# Autodesk Inventor assembly: Mount Setup
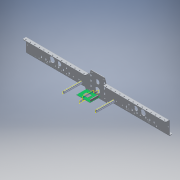
[picture p0: Inventor's stored thumbnail of the model, 180x180]
Saved by Autodesk Inventor 2017 (Build 210142000, 142)
## iProperties
Created: 2017-02-12
Part Number: Mount Setup
Document SubType Name: Assembly
Designer: Roksbot
Author: Roksbot
## Documents named in this file (4)
- C:\Users\Roksbot\Documents\Inventor\FRC ADIS16448\Mount Setup.iam
- C:\Users\Roksbot\Documents\Inventor\FRC ADIS16448\ADIS16448.ipt
- C:\Users\Roksbot\Documents\Inventor\FRC ADIS16448\am-2952a_AM14U3_Inside_Plate.ipt
- C:\Users\Roksbot\Documents\Inventor\FRC ADIS16448\3.875 Churo.ipt
## Components (4 placed, 3 different names)
1. ADIS16448:1 — Mate:1, Mate:2, Flush:2
2. am-2952a_AM14U3_Inside_Plate:1 — Insert:1, Insert:2, Mate:2
3. 3.875 Churo:1 — Insert:1, Flush:1, Mate:1, Mate:3, Mate:4
4. 3.875 Churo:2 — Insert:2, Flush:1, Mate:7, Mate:8
## Relationships (15: Mate 10, Insert 2, Flush 2, Symmetry 1)
- Insert:1: am-2952a_AM14U3_Inside_Plate:1 ↔ 3.875 Churo:1
- Insert:2: am-2952a_AM14U3_Inside_Plate:1 ↔ 3.875 Churo:2
- Flush:1: 3.875 Churo:1 ↔ 3.875 Churo:2
- Mate:1: ADIS16448:1 ↔ 3.875 Churo:1
- Mate:2 (25.4 mm): ADIS16448:1 ↔ am-2952a_AM14U3_Inside_Plate:1
- Mate:3: 3.875 Churo:1
- Mate:4: 3.875 Churo:1
- Mate:5
- Mate:6
- Mate:7: 3.875 Churo:2
- Mate:8: 3.875 Churo:2
- Mate:9
- Mate:10
- Symmetry:1
- Flush:2: ADIS16448:1
